# Autodesk Inventor assembly: Сборка
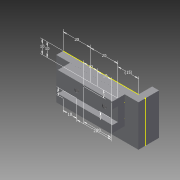
[picture p0: Inventor's stored thumbnail of the model, 180x180]
Saved by Autodesk Inventor 2015 (Build 190159000, 159)
## iProperties
Created: 2016-04-08
Part Number: Сборка
Document SubType Name: Assembly
Designer: Andreas
Author: Andreas
## Documents named in this file (4)
- C:\Users\criit\Desktop\ласт_ворк_v1.4\ласт_ворк_v1.1\ласт_ворк\проект\проект\левая каретка+деталь к ней\Сборка.iam
- C:\Users\criit\Desktop\ласт_ворк_v1.4\ласт_ворк_v1.1\ласт_ворк\проект\проект\левая каретка+деталь к ней\Karetka.ipt
- C:\Users\criit\Desktop\ласт_ворк_v1.4\ласт_ворк_v1.1\ласт_ворк\проект\проект\левая каретка+деталь к ней\detalKKoretke.ipt
- C:\Users\criit\Desktop\ласт_ворк_v1.4\ласт_ворк_v1.1\ласт_ворк\проект\проект\левая каретка+деталь к ней\Сборка\Design Accelerator\Bolted Connection1.iam
## Components (3 placed, 3 different names)
1. Karetka:1 — Rigid:1
2. detalKKoretke:1 — Rigid:1, Mate:1, Mate:2
3. Bolted Connection:1 [sub-assembly] — Mate:1, Mate:2
## Relationships (3: Mate 2, WeldJoint 1)
- Rigid:1 [WeldJoint]: Karetka:1 ↔ detalKKoretke:1
- Mate:1: detalKKoretke:1 ↔ Bolted Connection:1
- Mate:2: detalKKoretke:1 ↔ Bolted Connection:1
